# Autodesk Inventor assembly: Assembly shield 1
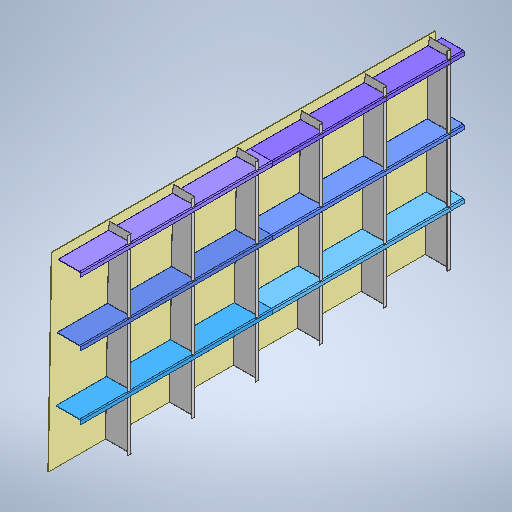
[picture p0: Inventor's stored thumbnail of the model, 512x512]
Saved by Autodesk Inventor 2026.2 (Build 302298000, 298)
## iProperties
Created: 2026-05-07
Part Number: Assembly shield 1
Document SubType Name: Assembly
Designer: admin
Author: admin
## Documents named in this file (6)
- C:\Users\admin\Documents\Inventor\GBK-Gubkinskiy\Assembly shield 1.iam
- C:\Users\admin\Documents\Inventor\GBK-Gubkinskiy\Part111.ipt
- C:\Users\admin\Documents\Inventor\GBK-Gubkinskiy\stringer 1.ipt
- C:\Users\admin\Documents\Inventor\GBK-Gubkinskiy\stringer 1.2.ipt
- C:\Users\admin\Documents\Inventor\GBK-Gubkinskiy\Part2.ipt
- C:\Users\admin\Documents\Inventor\GBK-Gubkinskiy\stringer 1.3.ipt
## Components (13 placed, 5 different names)
1. Part111:1
2. stringer 1:1
3. stringer 1.2:1
4. stringer 1:2
5. stringer 1.3:1
6. stringer 1.2:2
7. stringer 1.3:2
8. Part2:1
9. Part2:2
10. Part2:3
11. Part2:4
12. Part2:5
13. Part2:6
## Component patterns: (6 elements, first: Part2:1)
## Relationships (7: WeldJoint 6, Mate 1)
- [Mate]: Part111:1 ↔ Part2:1
- [WeldJoint] (2 mm): stringer 1:1 ↔ Part2:1
- [WeldJoint] (2 mm): stringer 1.2:1 ↔ Part2:1
- [WeldJoint]: stringer 1:1 ↔ stringer 1:2
- [WeldJoint] (2 mm): stringer 1.3:1 ↔ Part2:1
- [WeldJoint]: stringer 1.2:1 ↔ stringer 1.2:2
- [WeldJoint]: stringer 1.3:1 ↔ stringer 1.3:2
## Named parameters: d0_d6 = 0 mm
